# Autodesk Inventor assembly: Assembly1
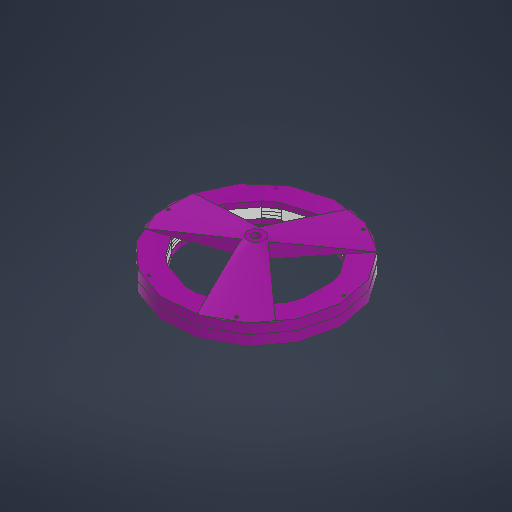
[picture p0: Inventor's stored thumbnail of the model, 512x512]
Saved by Autodesk Inventor 2025 (Build 290162010, 162A)
## iProperties
Created: 2024-11-09
Part Number: Assembly1
Document SubType Name: Assembly
Designer: river
Author: river
## Documents named in this file (10)
- C:\DATA\sem_08\Maquinas\proyecto\3d\Assembly1.iam
- C:\DATA\sem_08\Maquinas\proyecto\3d\lamina_estator.ipt
- C:\Users\river\Documents\Inventor\Content Center Files\R2025\en-US\DIN 625 SKF(4)\DIN 625 SKF - SKF 608-2Z.ipt
- C:\DATA\sem_08\Maquinas\proyecto\3d\rodamiento_shell.ipt
- C:\DATA\sem_08\Maquinas\proyecto\3d\perno.ipt
- C:\DATA\sem_08\Maquinas\proyecto\3d\lamina_rotor.ipt
- C:\DATA\sem_08\Maquinas\proyecto\3d\iman.ipt
- C:\DATA\sem_08\Maquinas\proyecto\3d\coil.ipt
- C:\DATA\sem_08\Maquinas\proyecto\3d\shell_1.ipt
- C:\DATA\sem_08\Maquinas\proyecto\3d\shell_base.ipt
## Components (35 placed, 9 different names)
1. lamina_estator:1 — Mate:1, Mate:2, Flush:1, Insert:1, Flush:2, Insert:6, Insert:7
2. lamina_estator:2 — Insert:1, Flush:2, Insert:2, Flush:3, Mate:7
3. lamina_estator:3 — Insert:2, Flush:3, Insert:4, Insert:5, Insert:10, Mate:8, Mate:9
4. DIN 625 SKF- with two Z shields SKF 608-2Z:1 — Insert:3, Insert:9
5. DIN 625 SKF- with two Z shields SKF 608-2Z:2 — Insert:3, Insert:8
6. rodamiento_shell:1 — Insert:4, Insert:5, Insert:8
7. rodamiento_shell:2 — Insert:6, Insert:7
8. perno:1 — Insert:9
9. lamina_rotor:1 — Mate:3, Flush:4, Flush:5
10. lamina_rotor:2 — Mate:3, Flush:4, Flush:5, Mate:4, Flush:6, Flush:7, Mate:5, Mate:6
11. lamina_rotor:3 — Mate:4, Flush:6, Flush:7, Insert:10
12. shell_1:1 — Insert:11, Insert:12
13. shell_base:1 — Mate:10, Mate:11, Mate:12, Insert:11, Insert:12
14. coil:1 — Mate:7, Mate:8, Mate:9
15. coil:2
16. coil:3
17. coil:4
18. coil:5
19. coil:6
20. coil:7
21. coil:8
22. coil:9
23. coil:10
24. coil:11
25. coil:12
26. iman:1 — Mate:5, Mate:6
27. iman:2
28. iman:3
29. iman:4
30. iman:5
31. iman:6 — Mate:10
32. iman:7 — Mate:11, Mate:12
33. iman:8
34. iman:9
35. iman:10
## Component patterns: (12 elements, first: coil:1), (10 elements, first: iman:1)
## Relationships (31: Mate 12, Insert 12, Flush 7)
- Mate:1: lamina_estator:1
- Mate:2: lamina_estator:1
- Flush:1: lamina_estator:1
- Insert:1: lamina_estator:1 ↔ lamina_estator:2
- Flush:2: lamina_estator:1 ↔ lamina_estator:2
- Insert:2: lamina_estator:2 ↔ lamina_estator:3
- Flush:3: lamina_estator:2 ↔ lamina_estator:3
- Insert:3: DIN 625 SKF- with two Z shields SKF 608-2Z:1 ↔ DIN 625 SKF- with two Z shields SKF 608-2Z:2
- Insert:4: lamina_estator:3 ↔ rodamiento_shell:1
- Insert:5: lamina_estator:3 ↔ rodamiento_shell:1
- Insert:6: lamina_estator:1 ↔ rodamiento_shell:2
- Insert:7: lamina_estator:1 ↔ rodamiento_shell:2
- Insert:8: DIN 625 SKF- with two Z shields SKF 608-2Z:2 ↔ rodamiento_shell:1
- Insert:9: DIN 625 SKF- with two Z shields SKF 608-2Z:1 ↔ perno:1
- Mate:3: lamina_rotor:1 ↔ lamina_rotor:2
- Flush:4: lamina_rotor:1 ↔ lamina_rotor:2
- Flush:5: lamina_rotor:1 ↔ lamina_rotor:2
- Mate:4: lamina_rotor:2 ↔ lamina_rotor:3
- Flush:6: lamina_rotor:2 ↔ lamina_rotor:3
- Flush:7: lamina_rotor:2 ↔ lamina_rotor:3
- Insert:10: lamina_estator:3 ↔ lamina_rotor:3
- Mate:5: lamina_rotor:2 ↔ iman:1
- Mate:6: lamina_rotor:2 ↔ iman:1
- Mate:7: lamina_estator:2 ↔ coil:1
- Mate:8: lamina_estator:3 ↔ coil:1
- Mate:9: lamina_estator:3 ↔ coil:1
- Mate:10: shell_base:1 ↔ iman:6
- Mate:11: shell_base:1 ↔ iman:7
- Mate:12: shell_base:1 ↔ iman:7
- Insert:11: shell_1:1 ↔ shell_base:1
- Insert:12: shell_1:1 ↔ shell_base:1
